# Autodesk Inventor assembly: Internal Cycloidal Actuator
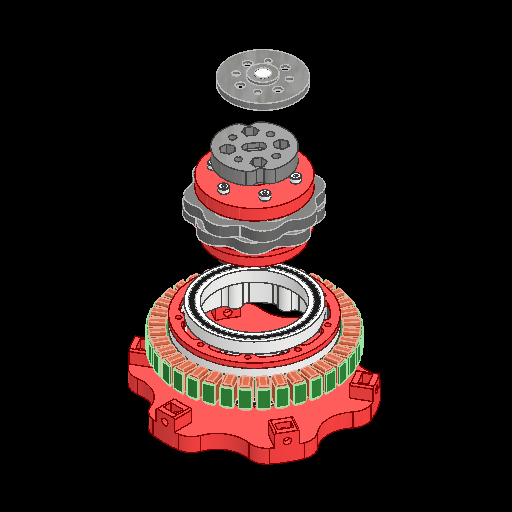
[picture p0: Inventor's stored thumbnail of the model, 512x512]
Saved by Autodesk Inventor 2025.2 (Build 292293000, 293)
## iProperties
Created: 2024-02-10
Part Number: Internal Cycloidal Actuator
Document SubType Name: Assembly
Designer: valer
Sending System: Autodesk Inventor 2023
Preprocessor: ST-DEVELOPER v19.2
Title: Internal Cycloidal Actuator.stp
Author: aaedm
## Documents named in this file (24)
- C:\Users\valer\Desktop\Cycloidal-BDLC\parts\Internal Cycloidal Actuator.iam
- C:\Users\valer\Desktop\Cycloidal-BDLC\parts\10010 Stator.ipt
- C:\Users\valer\Desktop\Cycloidal-BDLC\parts\Fixed_Ring.ipt
- C:\Users\valer\Desktop\Cycloidal-BDLC\parts\Cycloidal_Disk_1.ipt
- C:\Users\valer\Desktop\Cycloidal-BDLC\parts\Eccentric Shaft.ipt
- C:\Users\valer\Desktop\Cycloidal-BDLC\parts\Cycloidal_Disk_2.ipt
- C:\Users\valer\Desktop\Cycloidal-BDLC\parts\50x65x7mm_Bearing.ipt
- C:\Users\valer\Desktop\Cycloidal-BDLC\parts\Rotor.ipt
- C:\Users\valer\Desktop\Cycloidal-BDLC\parts\40x50x6mm_Bearing.ipt
- C:\Users\valer\Desktop\Cycloidal-BDLC\parts\Bottom_Housing.ipt
- Bottom_Housing.ipt
- C:\Users\valer\Desktop\Cycloidal-BDLC\parts\ODrive_S1.ipt
- C:\Users\valer\Desktop\Cycloidal-BDLC\parts\ODrive_S1_Cover.ipt
- C:\Users\valer\Desktop\Cycloidal-BDLC\parts\Top_Housing.ipt
- C:\Users\valer\Desktop\Cycloidal-BDLC\parts\M4_12mm_Screw.ipt
- C:\Users\valer\Desktop\Cycloidal-BDLC\parts\M3_8mm_Screw.ipt
- C:\Users\valer\Desktop\Cycloidal-BDLC\parts\M3_10mm_Screw.ipt
- C:\Users\valer\Desktop\Cycloidal-BDLC\parts\M3_Locknut.ipt
- C:\Users\valer\Desktop\Cycloidal-BDLC\parts\M3_35mm_Screw.ipt
- C:\Users\valer\Desktop\Cycloidal-BDLC\parts\Encoder_Holder.ipt
- C:\Users\valer\Desktop\Cycloidal-BDLC\parts\Housing_Spacer.ipt
- C:\Users\valer\Desktop\Cycloidal-BDLC\parts\8x2mm Magnet.ipt
- C:\Users\valer\Desktop\Cycloidal-BDLC\parts\Output Shaft.iam
- C:\Users\valer\Desktop\Cycloidal-BDLC\parts\12x21x5mm Bearing.ipt
## Components (58 placed, 22 different names)
1. 10010 Stator:1
2. Fixed_Ring:1
3. Cycloidal_Disk_1:1 — Mate:9, Mate:10
4. Eccentric_Shaft:1 — Mate:11, Mate:12, Mate:13, Mate:14, Mate:15, Mate:16, Mate:17, Mate:18
5. Cycloidal_Disk_2:1 — Mate:7, Mate:8
6. 50x65x7mm_Bearing:1
7. Rotor:1
8. 40x50x6mm_Bearing:1
9. Bottom_Housing:1
10. ODrive_S1:1
11. ODrive_S1_Cover:1
12. Top_Housing:1
13. M4_12mm_Screw:1
14. M4_12mm_Screw:2
15. M4_12mm_Screw:3
16. M4_12mm_Screw:4
17. M3_8mm_Screw:1
18. M3_8mm_Screw:2
19. M3_8mm_Screw:3
20. M3_8mm_Screw:4
21. M3_10mm_Screw:1
22. M3_10mm_Screw:2
23. M3_10mm_Screw:3
24. M3_10mm_Screw:4
25. M3_Locknut:1
26. M3_35mm_Screw:1
27. M3_Locknut:2
28. M3_35mm_Screw:2
29. M3_Locknut:3
30. M3_35mm_Screw:3
31. M3_Locknut:4
32. M3_35mm_Screw:4
33. M3_Locknut:5
34. M3_35mm_Screw:5
35. M3_Locknut:6
36. M3_35mm_Screw:6
37. M3_Locknut:7
38. M3_35mm_Screw:7
39. M3_Locknut:8
40. M3_35mm_Screw:8
41. M3_Locknut:9
42. M3_35mm_Screw:9
43. M4_12mm_Screw:5
44. M4_12mm_Screw:6
45. M4_12mm_Screw:7
46. M4_12mm_Screw:8
47. M4_12mm_Screw:9
48. M4_12mm_Screw:10
49. Encoder_Holder:1 — Mate:1, Mate:2, Mate:17, Mate:18
50. M4_12mm_Screw:11
51. M4_12mm_Screw:12
52. M4_12mm_Screw:13
53. M4_12mm_Screw:14
54. Housing_Spacer:1 — Mate:3
55. 8x2mm Magnet:1 — Mate:1, Mate:2
56. Output Shaft:1 [sub-assembly] — Mate:3, Mate:15, Mate:16
57. 12x21x5mm Bearing:1 — Mate:7, Mate:8, Mate:11, Mate:12
58. 12x21x5mm Bearing:2 — Mate:9, Mate:10, Mate:13, Mate:14
## Relationships (15: Mate 15)
- Mate:1: Encoder_Holder:1 ↔ 8x2mm Magnet:1
- Mate:2: Encoder_Holder:1 ↔ 8x2mm Magnet:1
- Mate:3: Housing_Spacer:1 ↔ Output Shaft:1
- Mate:7: Cycloidal_Disk_2:1 ↔ 12x21x5mm Bearing:1
- Mate:8: Cycloidal_Disk_2:1 ↔ 12x21x5mm Bearing:1
- Mate:9: Cycloidal_Disk_1:1 ↔ 12x21x5mm Bearing:2
- Mate:10: Cycloidal_Disk_1:1 ↔ 12x21x5mm Bearing:2
- Mate:11: Eccentric_Shaft:1 ↔ 12x21x5mm Bearing:1
- Mate:12: Eccentric_Shaft:1 ↔ 12x21x5mm Bearing:1
- Mate:13: Eccentric_Shaft:1 ↔ 12x21x5mm Bearing:2
- Mate:14: Eccentric_Shaft:1 ↔ 12x21x5mm Bearing:2
- Mate:15: Eccentric_Shaft:1 ↔ Output Shaft:1
- Mate:16: Eccentric_Shaft:1 ↔ Output Shaft:1
- Mate:17: Eccentric_Shaft:1 ↔ Encoder_Holder:1
- Mate:18: Eccentric_Shaft:1 ↔ Encoder_Holder:1
